# Autodesk Inventor assembly: LowerBody
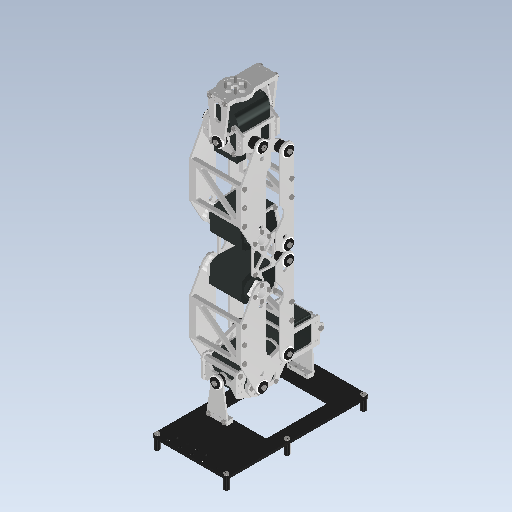
[picture p0: Inventor's stored thumbnail of the model, 512x512]
Saved by Autodesk Inventor 2020 (Build 240168000, 168)
## iProperties
Created: 2021-10-01
Part Number: LowerBody
Document SubType Name: Assembly
Designer: Masato
Mass: 1009.03 g
Surface Area: 2721.67 cm^2
Volume: 456.516 cm^3
Density: 2.21029 g/cm^3
Author: Masato
## Documents named in this file (13)
- C:\Users\Masato\Documents\Inventor\CIT Brains_Inventor\OpenPlatform_ver3_0\LowerBody\LowerBody.iam
- C:\Users\Masato\Documents\Inventor\CIT Brains_Inventor\OpenPlatform_ver3_0\LowerBody\Ankle\Ankle.iam
- C:\Users\Masato\Documents\Inventor\CIT Brains_Inventor\OpenPlatform_ver3_0\LowerBody\Ankle\Ankle_side_pitch.iam
- C:\Users\Masato\Documents\Inventor\CIT Brains_Inventor\OpenPlatform_ver3_0\LowerBody\Foot\Foot.iam
- C:\Users\Masato\Documents\Inventor\CIT Brains_Inventor\OpenPlatform_ver3_0\LowerBody\Knee\Knee.iam
- C:\Users\Masato\Documents\Inventor\CIT Brains_Inventor\OpenPlatform_ver3_0\LowerBody\Leg_joit\Leg_joint_roll_pitch.iam
- C:\Users\Masato\Documents\Inventor\CIT Brains_Inventor\OpenPlatform_ver3_0\LowerBody\Leg_joit\Leg_joint_roll_yaw.iam
- C:\Users\Masato\Documents\Inventor\CIT Brains_Inventor\OpenPlatform_ver3_0\LowerBody\Slider_crank\Slider_crank_mechanism.iam
- C:\Users\Masato\Documents\Inventor\CIT Brains_Inventor\OpenPlatform_ver3_0\LowerBody\Link\BackLink.iam
- C:\Users\Masato\Documents\Inventor\CIT Brains_Inventor\OpenPlatform_ver3_0\LowerBody\Link\FrontLink.iam
- C:\Users\Masato\Documents\Inventor\CIT Brains_Inventor\OpenPlatform_ver3_0\Ready_Made\Screw\M2_6-6.ipt
- C:\Users\Masato\Documents\Inventor\CIT Brains_Inventor\OpenPlatform_ver3_0\Ready_Made\Screw\M3-6.ipt
- C:\Users\Masato\Documents\Inventor\CIT Brains_Inventor\OpenPlatform_ver3_0\Ready_Made\Screw\M3-8.ipt
## Components (32 placed, 12 different names)
1. Ankle:1 [sub-assembly] — 挿入:15, 挿入:21, 挿入:22, 角度:11
2. Ankle_side_pitch:1 [sub-assembly] — 挿入:21, 挿入:23, 挿入:24, 挿入:25, 挿入:26, 挿入:35, 挿入:36, フラッシュ:5
3. Ankle_side_pitch:2 [sub-assembly] — 挿入:22, 挿入:27, 挿入:28, 挿入:29, 挿入:30, フラッシュ:5
4. Foot:1 [sub-assembly] — 挿入:15, 角度:3, 角度:5
5. Knee:1 [sub-assembly] — 挿入:31, 挿入:32, 挿入:33, 挿入:34
6. Leg_joint_roll_pitch:1 [sub-assembly] — 挿入:2, 挿入:37, 挿入:38, 角度:6, 角度:9, 角度:10, 挿入:70
7. Leg_joint_roll_yaw:1 [sub-assembly] — メイト:1, フラッシュ:3, フラッシュ:4, 角度:5, 角度:6, 挿入:69, 挿入:70
8. Slider_crank_mechanism:1 [sub-assembly] — 挿入:2, 挿入:69
9. BackLink:1 [sub-assembly] — 挿入:33, 挿入:36, 挿入:42, 挿入:46, 挿入:64, 挿入:66, 角度:7
10. FrontLink:1 [sub-assembly] — 挿入:31, 挿入:35, 角度:3, 挿入:63, 挿入:65, 角度:7, 角度:11, 角度:12
11. BackLink:2 [sub-assembly] — 挿入:34, 挿入:38, 挿入:39, 挿入:41, 挿入:44, 挿入:45, 角度:8
12. FrontLink:2 [sub-assembly] — 挿入:32, 挿入:37, 挿入:40, 挿入:43, 角度:8, 角度:10, 角度:12, 角度:9
13. M2_6-6:13 — 挿入:23
14. M2_6-6:14 — 挿入:24
15. M2_6-6:15 — 挿入:25
16. M2_6-6:16 — 挿入:26
17. M2_6-6:17 — 挿入:27
18. M2_6-6:18 — 挿入:28
19. M2_6-6:19 — 挿入:29
20. M2_6-6:20 — 挿入:30
21. M3-6:4 — 挿入:40
22. M3-6:5 — 挿入:39
23. M3-6:6 — 挿入:44
24. M3-6:7 — 挿入:43
25. M3-6:8 — 挿入:41
26. M3-6:9 — 挿入:45
27. M3-6:10 — 挿入:42
28. M3-6:11 — 挿入:46
29. M3-8:1 — 挿入:63
30. M3-8:2 — 挿入:64
31. M3-8:3 — 挿入:66
32. M3-8:4 — 挿入:65
## Relationships (47: Insert 34, Angle 9, Flush 3, Mate 1)
- メイト:1 [Mate]: Leg_joint_roll_yaw:1
- フラッシュ:3 [Flush]: Leg_joint_roll_yaw:1
- フラッシュ:4 [Flush]: Leg_joint_roll_yaw:1
- 挿入:2 [Insert]: Leg_joint_roll_pitch:1 ↔ Slider_crank_mechanism:1
- 挿入:15 [Insert]: Ankle:1 ↔ Foot:1
- 挿入:21 [Insert]: Ankle:1 ↔ Ankle_side_pitch:1
- 挿入:22 [Insert]: Ankle:1 ↔ Ankle_side_pitch:2
- 挿入:23 [Insert]: Ankle_side_pitch:1 ↔ M2_6-6:13
- 挿入:24 [Insert]: Ankle_side_pitch:1 ↔ M2_6-6:14
- 挿入:25 [Insert]: Ankle_side_pitch:1 ↔ M2_6-6:15
- 挿入:26 [Insert]: Ankle_side_pitch:1 ↔ M2_6-6:16
- 挿入:27 [Insert]: Ankle_side_pitch:2 ↔ M2_6-6:17
- 挿入:28 [Insert]: Ankle_side_pitch:2 ↔ M2_6-6:18
- 挿入:29 [Insert]: Ankle_side_pitch:2 ↔ M2_6-6:19
- 挿入:30 [Insert]: Ankle_side_pitch:2 ↔ M2_6-6:20
- 挿入:31 [Insert]: Knee:1 ↔ FrontLink:1
- 挿入:32 [Insert]: Knee:1 ↔ FrontLink:2
- 挿入:33 [Insert]: Knee:1 ↔ BackLink:1
- 挿入:34 [Insert]: Knee:1 ↔ BackLink:2
- 挿入:35 [Insert]: Ankle_side_pitch:1 ↔ FrontLink:1
- 挿入:36 [Insert]: Ankle_side_pitch:1 ↔ BackLink:1
- 挿入:37 [Insert]: Leg_joint_roll_pitch:1 ↔ FrontLink:2
- 挿入:38 [Insert]: Leg_joint_roll_pitch:1 ↔ BackLink:2
- 角度:3 [Angle] (0 deg): Foot:1 ↔ FrontLink:1
- 角度:5 [Angle] (0 deg): Foot:1 ↔ Leg_joint_roll_yaw:1
- 挿入:39 [Insert]: BackLink:2 ↔ M3-6:5
- 挿入:40 [Insert]: FrontLink:2 ↔ M3-6:4
- 挿入:41 [Insert]: BackLink:2 ↔ M3-6:8
- 挿入:42 [Insert]: BackLink:1 ↔ M3-6:10
- 挿入:43 [Insert]: FrontLink:2 ↔ M3-6:7
- 挿入:44 [Insert]: BackLink:2 ↔ M3-6:6
- 挿入:45 [Insert]: BackLink:2 ↔ M3-6:9
- 挿入:46 [Insert]: BackLink:1 ↔ M3-6:11
- 挿入:63 [Insert]: FrontLink:1 ↔ M3-8:1
- 挿入:64 [Insert]: BackLink:1 ↔ M3-8:2
- 挿入:65 [Insert]: FrontLink:1 ↔ M3-8:4
- 挿入:66 [Insert]: BackLink:1 ↔ M3-8:3
- フラッシュ:5 [Flush]: Ankle_side_pitch:1 ↔ Ankle_side_pitch:2
- 角度:6 [Angle] (0 deg): Leg_joint_roll_pitch:1 ↔ Leg_joint_roll_yaw:1
- 角度:7 [Angle] (0 deg): BackLink:1 ↔ FrontLink:1
- 角度:8 [Angle] (0 deg): BackLink:2 ↔ FrontLink:2
- 角度:9 [Angle] (0 deg): Leg_joint_roll_pitch:1 ↔ FrontLink:2
- 角度:10 [Angle] (0 deg): Leg_joint_roll_pitch:1 ↔ FrontLink:2
- 角度:11 [Angle] (0 deg): Ankle:1 ↔ FrontLink:1
- 角度:12 [Angle] (0 deg): FrontLink:1 ↔ FrontLink:2
- 挿入:69 [Insert]: Leg_joint_roll_yaw:1 ↔ Slider_crank_mechanism:1
- 挿入:70 [Insert]: Leg_joint_roll_pitch:1 ↔ Leg_joint_roll_yaw:1
